# Autodesk Inventor assembly: Pannels Assembly V2
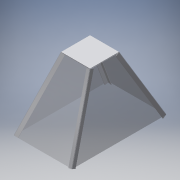
[picture p0: Inventor's stored thumbnail of the model, 180x180]
Saved by Autodesk Inventor 2016 (Build 200138000, 138)
## iProperties
Created: 2018-06-14
Part Number: Pannels Assembly V2
Document SubType Name: Assembly
Designer: dwpbe
Author: dwpbe
## Documents named in this file (5)
- F:\Robotics\Off Season\Blannon\Pannels Assembly V2.iam
- F:\Robotics\Off Season\Blannon\Polycarb Side1 Pannel.ipt
- F:\Robotics\Off Season\Blannon\Polycarb Front Pannel.ipt
- F:\Robotics\Off Season\Blannon\Turntable Bottom.ipt
- F:\Robotics\Off Season\Blannon\AngleL.ipt
## Components (9 placed, 4 different names)
1. Turntable Bottom:1 — Mate:25, Mate:26, Mate:27, Mate:28
2. AngleL:1 — Mate:29, Mate:30
3. AngleL:2 — Mate:31, Mate:32
4. AngleL:3 — Mate:33, Mate:34
5. AngleL:4 — Mate:35, Mate:36
6. Polycarb Side1 Pannel:1 — Mate:10, Mate:15, Mate:21, Mate:22, Mate:27, Mate:29, Mate:35
7. Polycarb Side1 Pannel:2 — Mate:13, Mate:14, Mate:23, Mate:24, Mate:31, Mate:33
8. Polycarb Front Pannel:1 — Mate:12, Mate:19, Mate:21, Mate:24, Mate:28, Mate:34, Mate:36
9. Polycarb Front Pannel:2 — Mate:9, Mate:20, Mate:22, Mate:23, Mate:30, Mate:32
## Relationships (24: Mate 24)
- Mate:9: Polycarb Front Pannel:2
- Mate:10: Polycarb Side1 Pannel:1
- Mate:12: Polycarb Front Pannel:1
- Mate:13: Polycarb Side1 Pannel:2
- Mate:14 (-203.2 mm): Polycarb Side1 Pannel:2
- Mate:15 (203.2 mm): Polycarb Side1 Pannel:1
- Mate:19 (330.2 mm): Polycarb Front Pannel:1
- Mate:20 (-330.2 mm): Polycarb Front Pannel:2
- Mate:21: Polycarb Side1 Pannel:1 ↔ Polycarb Front Pannel:1
- Mate:22: Polycarb Side1 Pannel:1 ↔ Polycarb Front Pannel:2
- Mate:23: Polycarb Side1 Pannel:2 ↔ Polycarb Front Pannel:2
- Mate:24: Polycarb Side1 Pannel:2 ↔ Polycarb Front Pannel:1
- Mate:25 (-101.6 mm): Turntable Bottom:1
- Mate:26 (-101.6 mm): Turntable Bottom:1
- Mate:27: Turntable Bottom:1 ↔ Polycarb Side1 Pannel:1
- Mate:28: Turntable Bottom:1 ↔ Polycarb Front Pannel:1
- Mate:29: AngleL:1 ↔ Polycarb Side1 Pannel:1
- Mate:30: AngleL:1 ↔ Polycarb Front Pannel:2
- Mate:31: AngleL:2 ↔ Polycarb Side1 Pannel:2
- Mate:32: AngleL:2 ↔ Polycarb Front Pannel:2
- Mate:33: AngleL:3 ↔ Polycarb Side1 Pannel:2
- Mate:34: AngleL:3 ↔ Polycarb Front Pannel:1
- Mate:35: AngleL:4 ↔ Polycarb Side1 Pannel:1
- Mate:36: AngleL:4 ↔ Polycarb Front Pannel:1
